# Autodesk Inventor assembly: Completa
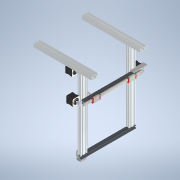
[picture p0: Inventor's stored thumbnail of the model, 180x180]
Saved by Autodesk Inventor 2021 (Build 250183000, 183)
## iProperties
Created: 2023-01-20
Part Number: Completa
Document SubType Name: Assembly
Designer: Diego.labarca
Author: Diego.labarca
## Documents named in this file (14)
- E:\Dropbox\Inventor\Impresora 3D\Arreglos Impresora\IDEX\Completa.iam
- E:\Dropbox\Inventor\Impresora 3D\Arreglos Impresora\IDEX\2040x435.ipt
- E:\Dropbox\Inventor\Impresora 3D\Arreglos Impresora\IDEX\2040x350.ipt
- E:\Dropbox\Inventor\Impresora 3D\Arreglos Impresora\IDEX\2020x330.ipt
- E:\Dropbox\Inventor\Impresora 3D\Arreglos Impresora\IDEX\MGN9x350.ipt
- E:\Dropbox\Inventor\Impresora 3D\Arreglos Impresora\IDEX\MGN9H.ipt
- E:\Dropbox\Inventor\Impresora 3D\Arreglos Impresora\IDEX\Nema17.ipt
- E:\Dropbox\Inventor\Impresora 3D\Arreglos Impresora\IDEX\Pulley GT2 20T 5ID.ipt
- E:\Dropbox\Inventor\Impresora 3D\Arreglos Impresora\IDEX\Idler GT2 20T 3ID.ipt
- E:\Dropbox\Inventor\Impresora 3D\Arreglos Impresora\IDEX\Soporte Idler Z.ipt
- E:\Dropbox\Inventor\Impresora 3D\Arreglos Impresora\IDEX\Soporte Linear Rail X.ipt
- E:\Dropbox\Inventor\Impresora 3D\Arreglos Impresora\IDEX\MGN12x350.ipt
- E:\Dropbox\Inventor\Impresora 3D\Arreglos Impresora\IDEX\MGN12H.ipt
- E:\Dropbox\Inventor\Impresora 3D\Arreglos Impresora\IDEX\Base Motor X1.ipt
## Components (21 placed, 13 different names)
1. 2020x330:1 — Nivelación:4, Nivelación:5, Coincidencia:2, Coincidencia:9, Nivelación:9, Nivelación:10, Nivelación:12
2. MGN9x350:1 — Coincidencia:4, Coincidencia:5, Coincidencia:10, Coincidencia:11
3. MGN9H:1 — Coincidencia:5, Coincidencia:10, Nivelación:11, Insertar:2, Insertar:3
4. Nema17:1 — Coincidencia:6, Ángulo:1, Coincidencia:15
5. Pulley GT2 20T 5ID:1 — Nivelación:8, Coincidencia:15
6. Idler GT2 20T 3ID:1 — Nivelación:8, Insertar:1
7. Soporte Idler Z:1 — Coincidencia:9, Nivelación:9, Nivelación:10, Insertar:1
8. 2020x330:2 — Nivelación:12, Coincidencia:12, Coincidencia:13, Coincidencia:16, Nivelación:17, Coincidencia:17, Coincidencia:23, Nivelación:24, Nivelación:28, Coincidencia:27
9. Soporte Linear Rail X:1 — Insertar:2, Insertar:3, Coincidencia:13
10. MGN12x350:1 — Coincidencia:16, Nivelación:17, Coincidencia:17, Coincidencia:18, Coincidencia:19, Nivelación:18, Nivelación:21
11. MGN12H:1 — Coincidencia:18, Coincidencia:19, Nivelación:18, Nivelación:19, Nivelación:20, Coincidencia:20
12. MGN12H:2 — Nivelación:19, Nivelación:20, Coincidencia:20, Nivelación:21
13. Nema17:2 — Nivelación:26, Coincidencia:24, Coincidencia:26, Nivelación:28, Insertar:4, Insertar:5
14. Pulley GT2 20T 5ID:2 — Nivelación:27, Coincidencia:24
15. Nema17:3 — Coincidencia:23, Nivelación:24, Nivelación:25, Nivelación:26, Coincidencia:28
16. Pulley GT2 20T 5ID:4 — Nivelación:27, Coincidencia:27, Coincidencia:28
17. Base Motor X1:1 — Insertar:4, Insertar:5
18. 2040x350:1 — Coincidencia:1, Nivelación:1, Nivelación:2, Coincidencia:4, Coincidencia:6, Ángulo:1
19. 2040x435:1 — Coincidencia:1, Nivelación:1, Nivelación:2, Nivelación:3, Coincidencia:11, Nivelación:11, Coincidencia:12, Nivelación:25
20. 2040x350:2
21. 2040x435:2 — Nivelación:4, Nivelación:5, Coincidencia:2, Coincidencia:26
## Component patterns: (2 elements, first: 2040x350:1 + 2040x435:1)
## Relationships (47: Mate 21, Flush 20, Insert 5, Angle 1)
- Coincidencia:1 [Mate]: 2040x350:1 ↔ 2040x435:1
- Nivelación:1 [Flush]: 2040x350:1 ↔ 2040x435:1
- Nivelación:2 [Flush] (-65 mm): 2040x350:1 ↔ 2040x435:1
- Nivelación:3 [Flush] (-125 mm): 2040x435:1
- Nivelación:4 [Flush]: 2020x330:1 ↔ 2040x435:2
- Nivelación:5 [Flush]: 2020x330:1 ↔ 2040x435:2
- Coincidencia:2 [Mate]: 2020x330:1 ↔ 2040x435:2
- Coincidencia:4 [Mate] (50 mm): MGN9x350:1 ↔ 2040x350:1
- Coincidencia:5 [Mate]: MGN9x350:1 ↔ MGN9H:1
- Coincidencia:6 [Mate]: Nema17:1 ↔ 2040x350:1
- Nivelación:8 [Flush]: Pulley GT2 20T 5ID:1 ↔ Idler GT2 20T 3ID:1
- Ángulo:1 [Angle] (0 deg): Nema17:1 ↔ 2040x350:1
- Coincidencia:9 [Mate]: 2020x330:1 ↔ Soporte Idler Z:1
- Nivelación:9 [Flush]: 2020x330:1 ↔ Soporte Idler Z:1
- Nivelación:10 [Flush]: 2020x330:1 ↔ Soporte Idler Z:1
- Insertar:1 (1 mm): Idler GT2 20T 3ID:1 ↔ Soporte Idler Z:1
- Coincidencia:10 [Mate]: MGN9x350:1 ↔ MGN9H:1
- Coincidencia:11 [Mate]: MGN9x350:1 ↔ 2040x435:1
- Nivelación:11 [Flush]: MGN9H:1 ↔ 2040x435:1
- Nivelación:12 [Flush]: 2020x330:1 ↔ 2020x330:2
- Coincidencia:12 [Mate] (2 mm): 2020x330:2 ↔ 2040x435:1
- Insertar:2: MGN9H:1 ↔ Soporte Linear Rail X:1
- Insertar:3: MGN9H:1 ↔ Soporte Linear Rail X:1
- Coincidencia:13 [Mate]: 2020x330:2 ↔ Soporte Linear Rail X:1
- Coincidencia:15 [Mate]: Nema17:1 ↔ Pulley GT2 20T 5ID:1
- Coincidencia:16 [Mate]: 2020x330:2 ↔ MGN12x350:1
- Nivelación:17 [Flush] (-10 mm): 2020x330:2 ↔ MGN12x350:1
- Coincidencia:17 [Mate]: 2020x330:2 ↔ MGN12x350:1
- Coincidencia:18 [Mate]: MGN12x350:1 ↔ MGN12H:1
- Coincidencia:19 [Mate]: MGN12x350:1 ↔ MGN12H:1
- Nivelación:18 [Flush]: MGN12x350:1 ↔ MGN12H:1
- Nivelación:19 [Flush]: MGN12H:1 ↔ MGN12H:2
- Nivelación:20 [Flush]: MGN12H:1 ↔ MGN12H:2
- Coincidencia:20 [Mate]: MGN12H:1 ↔ MGN12H:2
- Nivelación:21 [Flush]: MGN12x350:1 ↔ MGN12H:2
- Coincidencia:23 [Mate] (5 mm): 2020x330:2 ↔ Nema17:3
- Nivelación:24 [Flush] (-2 mm): 2020x330:2 ↔ Nema17:3
- Nivelación:25 [Flush] (2 mm): Nema17:3 ↔ 2040x435:1
- Nivelación:26 [Flush]: Nema17:2 ↔ Nema17:3
- Nivelación:27 [Flush]: Pulley GT2 20T 5ID:2 ↔ Pulley GT2 20T 5ID:4
- Coincidencia:24 [Mate]: Nema17:2 ↔ Pulley GT2 20T 5ID:2
- Coincidencia:26 [Mate] (5 mm): Nema17:2 ↔ 2040x435:2
- Nivelación:28 [Flush] (2 mm): 2020x330:2 ↔ Nema17:2
- Coincidencia:27 [Mate] (3.5 mm): 2020x330:2 ↔ Pulley GT2 20T 5ID:4
- Coincidencia:28 [Mate]: Nema17:3 ↔ Pulley GT2 20T 5ID:4
- Insertar:4: Nema17:2 ↔ Base Motor X1:1
- Insertar:5: Nema17:2 ↔ Base Motor X1:1
